# Autodesk Inventor assembly: gyroMergedWheelBody
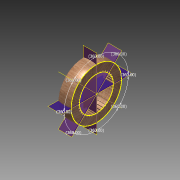
[picture p0: Inventor's stored thumbnail of the model, 180x180]
Saved by Autodesk Inventor 2013 (Build 170138000, 138)
## iProperties
Created: 2013-01-23
Part Number: gyroMergedWheelBody
Document SubType Name: Assembly
Designer: Nano
Author: Nano
## Documents named in this file (2)
- C:\Users\Nano\Documents\InventorByron\InventorMasterProject\gyroPhone01\gyroMergedWheelBody.iam
- C:\Users\Nano\Documents\InventorByron\InventorMasterProject\gyroPhone01\bigWheelWedge01.ipt
## Components (8 placed, 1 different names)
1. bigWheelWedge01:1
2. bigWheelWedge01:2
3. bigWheelWedge01:3
4. bigWheelWedge01:4
5. bigWheelWedge01:5
6. bigWheelWedge01:6
7. bigWheelWedge01:7
8. bigWheelWedge01:8
## Component patterns: (8 elements, first: bigWheelWedge01:1)
